# Autodesk Inventor assembly: Attempt 1
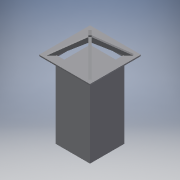
[picture p0: Inventor's stored thumbnail of the model, 180x180]
Saved by Autodesk Inventor 2019.1 (Build 231200000, 200)
## iProperties
Created: 2020-12-23
Part Number: Attempt 1
Document SubType Name: Assembly
Designer: Thomas Dodd
Author: Thomas Dodd
## Documents named in this file (5)
- C:\Users\Thomas Dodd\Desktop\Joachim's Project\Attempt 1.iam
- C:\Users\Thomas Dodd\Desktop\Joachim's Project\Box.ipt
- C:\Users\Thomas Dodd\Desktop\Joachim's Project\Lower Base Plate.ipt
- C:\Users\Thomas Dodd\Desktop\Joachim's Project\Upper Base Plate.ipt
- C:\Users\Thomas Dodd\Desktop\Joachim's Project\Main Beam.ipt
## Components (13 placed, 4 different names)
1. Box:1 — Mate:1, Mate:2, Mate:3, Mate:4
2. Lower Base Plate:5 — Rigid:3
3. Lower Base Plate:6 — Rigid:1, Rigid:2, Mate:1
4. Lower Base Plate:7 — Rigid:2, Mate:2, Mate:5
5. Lower Base Plate:8 — Rigid:1, Rigid:3
6. Upper Base Plate:1 — Rigid:6
7. Upper Base Plate:2 — Rigid:5, Mate:5, Mate:10, Flush:2
8. Upper Base Plate:3 — Rigid:4, Rigid:5, Mate:4, Mate:6, Mate:7, Mate:8, Mate:9
9. Upper Base Plate:4 — Rigid:4, Rigid:6, Mate:3, Flush:1, Mate:11
10. Main Beam:1 — Mate:6, Mate:11, Mate:13
11. Main Beam:2 — Mate:7, Flush:1, Mate:12
12. Main Beam:3 — Mate:8, Mate:10, Mate:13
13. Main Beam:4 — Mate:9, Flush:2, Mate:12
## Relationships (21: Mate 13, WeldJoint 6, Flush 2)
- Rigid:1 [WeldJoint]: Lower Base Plate:6 ↔ Lower Base Plate:8
- Rigid:2 [WeldJoint]: Lower Base Plate:6 ↔ Lower Base Plate:7
- Rigid:3 [WeldJoint]: Lower Base Plate:5 ↔ Lower Base Plate:8
- Mate:1: Box:1 ↔ Lower Base Plate:6
- Mate:2: Box:1 ↔ Lower Base Plate:7
- Rigid:4 [WeldJoint]: Upper Base Plate:3 ↔ Upper Base Plate:4
- Rigid:5 [WeldJoint]: Upper Base Plate:2 ↔ Upper Base Plate:3
- Rigid:6 [WeldJoint]: Upper Base Plate:1 ↔ Upper Base Plate:4
- Mate:3: Box:1 ↔ Upper Base Plate:4
- Mate:4: Box:1 ↔ Upper Base Plate:3
- Mate:5: Lower Base Plate:7 ↔ Upper Base Plate:2
- Mate:6: Upper Base Plate:3 ↔ Main Beam:1
- Mate:7: Upper Base Plate:3 ↔ Main Beam:2
- Mate:8: Upper Base Plate:3 ↔ Main Beam:3
- Mate:9: Upper Base Plate:3 ↔ Main Beam:4
- Flush:1 (-20 mm): Upper Base Plate:4 ↔ Main Beam:2
- Mate:10 (-20 mm): Upper Base Plate:2 ↔ Main Beam:3
- Mate:11 (-20 mm): Upper Base Plate:4 ↔ Main Beam:1
- Flush:2 (-20 mm): Upper Base Plate:2 ↔ Main Beam:4
- Mate:12 (40 mm): Main Beam:2 ↔ Main Beam:4
- Mate:13 (40 mm): Main Beam:1 ↔ Main Beam:3
